# Autodesk Inventor assembly: Assembly1
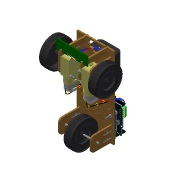
[picture p0: Inventor's stored thumbnail of the model, 180x180]
Saved by Autodesk Inventor 2016 (Build 200138000, 138)
## iProperties
Created: 2014-07-12
Part Number: Assembly1
Document SubType Name: Assembly
Designer: Sebastian
Author: Sebastian
## Documents named in this file (18)
- C:\Users\Sebastian\Dropbox\Projects\ERNIE\3D\Assembly1.iam
- C:\Users\Sebastian\Dropbox\Projects\ERNIE\3D\base.ipt
- C:\Users\Sebastian\Dropbox\Projects\ERNIE\3D\wheel.ipt
- C:\Users\Sebastian\Dropbox\Projects\ERNIE\3D\axel mount (3mm shaft).ipt
- C:\Users\Sebastian\Dropbox\Projects\ERNIE\3D\shaft.ipt
- C:\Users\Sebastian\Dropbox\Projects\ERNIE\3D\Imported Components\arduino uno\arduino uno.iam
- C:\Users\Sebastian\Dropbox\Projects\ERNIE\3D\servo.iam
- C:\Users\Sebastian\Dropbox\Projects\ERNIE\3D\motor mount.iam
- C:\Users\Sebastian\Dropbox\Projects\ERNIE\3D\motor mount - right.iam
- C:\Users\Sebastian\Dropbox\Projects\ERNIE\3D\m3 20mm screw.ipt
- C:\Users\Sebastian\Dropbox\Projects\ERNIE\3D\3mm nut.ipt
- C:\Users\Sebastian\Dropbox\Projects\ERNIE\3D\Sensor Holder.ipt
- C:\Users\Sebastian\Dropbox\Projects\ERNIE\3D\Imported Components\motor shield\Motor Shield V2.iam
- C:\Users\Sebastian\Dropbox\Projects\ERNIE\3D\pcb.ipt
- C:\Users\Sebastian\Dropbox\Projects\ERNIE\3D\Assembly1\AIP\Cable and Harness\Assembly1.Harness2.iam
- C:\Users\Sebastian\Dropbox\Projects\ERNIE\3D\6AA Battery Pack.ipt
- C:\Users\Sebastian\Dropbox\Projects\ERNIE\3D\Assembly1\AIP\Cable and Harness\Assembly1.Harness3.iam
- C:\Users\Sebastian\Dropbox\Projects\ERNIE\3D\BatteryDone.ipt
## Components (44 placed, 17 different names)
1. base:2 — Flush:6, Mate:11, Mate:12, Flush:7, Mate:13, Mate:14, Flush:8, Flush:9, Mate:15, Mate:16, Mate:17, Mate:18, Mate:19, Mate:20, Mate:21, Mate:22, Mate:23, Mate:24, Mate:25, Mate:26, Mate:27, Mate:28, Mate:29, Mate:30, Mate:31, Mate:32, Mate:33, Mate:34, Mate:45, Mate:56, Mate:65, Mate:68, Mate:69, Mate:70, Mate:71, Mate:72, Mate:73, Mate:74, Mate:75
2. axel mount (3mm shaft):2 — Flush:6, Mate:11, Mate:12
3. axel mount (3mm shaft):1 — Flush:7, Mate:13, Mate:14, Mate:43, Flush:10
4. arduino uno:1 [sub-assembly] — Mate:45, Mate:48, Mate:49, Mate:53, Mate:56, Mate:59, Mate:67
5. shaft:1 — Mate:43, Flush:10, Mate:44
6. wheel:1 — Mate:44
7. wheel:2
8. wheel:3
9. servo:1 [sub-assembly] — Mate:69
10. motor mount:1 [sub-assembly] — Flush:9, Mate:17, Mate:18
11. motor mount - right:1 [sub-assembly] — Flush:8, Mate:15, Mate:16
12. m3 20mm screw:1 — Mate:22, Mate:31, Mate:35
13. m3 20mm screw:2 — Mate:23, Mate:27, Mate:42
14. m3 20mm screw:3 — Mate:24, Mate:32, Mate:41
15. m3 20mm screw:4 — Mate:25, Mate:29, Mate:37
16. m3 20mm screw:5 — Mate:26, Mate:28, Mate:38
17. m3 20mm screw:6 — Mate:21, Mate:30, Mate:36
18. m3 20mm screw:7 — Mate:20, Mate:33, Mate:39
19. m3 20mm screw:8 — Mate:19, Mate:34, Mate:40
20. 3mm nut:1 — Mate:36
21. 3mm nut:2 — Mate:35
22. 3mm nut:3 — Mate:40
23. 3mm nut:4 — Mate:39
24. 3mm nut:5 — Mate:41
25. 3mm nut:6 — Mate:38
26. 3mm nut:7 — Mate:37
27. 3mm nut:8 — Mate:42
28. m3 20mm screw:9 — Mate:67, Mate:68
29. m3 20mm screw:10 — Mate:48, Mate:49, Mate:52, Mate:55, Mate:64
30. 3mm nut:9 — Mate:54, Mate:55
31. 3mm nut:10 — Mate:52, Mate:53, Mate:54
32. 3mm nut:11 — Mate:59, Mate:61
33. 3mm nut:12 — Mate:61
34. 3mm nut:14 — Mate:64, Mate:65
35. Sensor Holder:1 — Mate:73, Mate:74, Mate:75, Mate:78
36. Sensor Holder:2 — Mate:70, Mate:71, Mate:72, Mate:76, Mate:77, Mate:79
37. Motor Shield V2:1 [sub-assembly]
38. pcb:1 — Mate:76, Mate:77, Mate:78, Mate:79
39. 6AA Battery Pack:1
40. Harness2 [sub-assembly]
41. Harness3 [sub-assembly]
42. BatteryDone:1
43. BatteryDone:2
44. BatteryDone:3
## Relationships (64: Mate 59, Flush 5)
- Flush:6: base:2 ↔ axel mount (3mm shaft):2
- Mate:11: base:2 ↔ axel mount (3mm shaft):2
- Mate:12: base:2 ↔ axel mount (3mm shaft):2
- Flush:7: base:2 ↔ axel mount (3mm shaft):1
- Mate:13: base:2 ↔ axel mount (3mm shaft):1
- Mate:14: base:2 ↔ axel mount (3mm shaft):1
- Flush:8: base:2 ↔ motor mount - right:1
- Flush:9: base:2 ↔ motor mount:1
- Mate:15: base:2 ↔ motor mount - right:1
- Mate:16: base:2 ↔ motor mount - right:1
- Mate:17: base:2 ↔ motor mount:1
- Mate:18: base:2 ↔ motor mount:1
- Mate:19: base:2 ↔ m3 20mm screw:8
- Mate:20: base:2 ↔ m3 20mm screw:7
- Mate:21: base:2 ↔ m3 20mm screw:6
- Mate:22: base:2 ↔ m3 20mm screw:1
- Mate:23: base:2 ↔ m3 20mm screw:2
- Mate:24: base:2 ↔ m3 20mm screw:3
- Mate:25: base:2 ↔ m3 20mm screw:4
- Mate:26: base:2 ↔ m3 20mm screw:5
- Mate:27: base:2 ↔ m3 20mm screw:2
- Mate:28: base:2 ↔ m3 20mm screw:5
- Mate:29: base:2 ↔ m3 20mm screw:4
- Mate:30: base:2 ↔ m3 20mm screw:6
- Mate:31: base:2 ↔ m3 20mm screw:1
- Mate:32: base:2 ↔ m3 20mm screw:3
- Mate:33: base:2 ↔ m3 20mm screw:7
- Mate:34: base:2 ↔ m3 20mm screw:8
- Mate:35: m3 20mm screw:1 ↔ 3mm nut:2
- Mate:36: m3 20mm screw:6 ↔ 3mm nut:1
- Mate:37: m3 20mm screw:4 ↔ 3mm nut:7
- Mate:38: m3 20mm screw:5 ↔ 3mm nut:6
- Mate:39: m3 20mm screw:7 ↔ 3mm nut:4
- Mate:40: m3 20mm screw:8 ↔ 3mm nut:3
- Mate:41: m3 20mm screw:3 ↔ 3mm nut:5
- Mate:42: m3 20mm screw:2 ↔ 3mm nut:8
- Mate:43: axel mount (3mm shaft):1 ↔ shaft:1
- Flush:10 (4 mm): axel mount (3mm shaft):1 ↔ shaft:1
- Mate:44: shaft:1 ↔ wheel:1
- Mate:45: base:2 ↔ arduino uno:1
- Mate:48: arduino uno:1 ↔ m3 20mm screw:10
- Mate:49: arduino uno:1 ↔ m3 20mm screw:10
- Mate:52: m3 20mm screw:10 ↔ 3mm nut:10
- Mate:53: arduino uno:1 ↔ 3mm nut:10
- Mate:54: 3mm nut:9 ↔ 3mm nut:10
- Mate:55: m3 20mm screw:10 ↔ 3mm nut:9
- Mate:56 (5 mm): base:2 ↔ arduino uno:1
- Mate:59: arduino uno:1 ↔ 3mm nut:11
- Mate:61: 3mm nut:11 ↔ 3mm nut:12
- Mate:64: m3 20mm screw:10 ↔ 3mm nut:14
- Mate:65: base:2 ↔ 3mm nut:14
- Mate:67: arduino uno:1 ↔ m3 20mm screw:9
- Mate:68: base:2 ↔ m3 20mm screw:9
- Mate:69: base:2 ↔ servo:1
- Mate:70: base:2 ↔ Sensor Holder:2
- Mate:71: base:2 ↔ Sensor Holder:2
- Mate:72: base:2 ↔ Sensor Holder:2
- Mate:73: base:2 ↔ Sensor Holder:1
- Mate:74: base:2 ↔ Sensor Holder:1
- Mate:75: base:2 ↔ Sensor Holder:1
- Mate:76: Sensor Holder:2 ↔ pcb:1
- Mate:77: Sensor Holder:2 ↔ pcb:1
- Mate:78: Sensor Holder:1 ↔ pcb:1
- Mate:79: Sensor Holder:2 ↔ pcb:1
